# Autodesk Inventor assembly: Flash Hobby D3530 1100KV
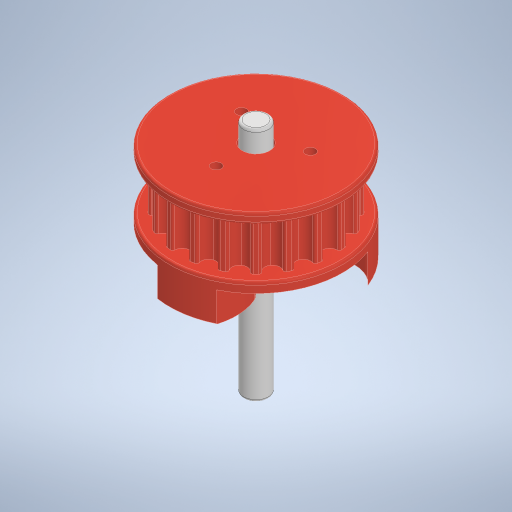
[picture p0: Inventor's stored thumbnail of the model, 512x512]
Saved by Autodesk Inventor 2023.2 (Build 272271000, 271)
## iProperties
Created: 2022-12-15
Part Number: Flash Hobby D3530 1100KV
Document SubType Name: Assembly
Designer: Nathan Cai
Author: Nathan Cai
## Documents named in this file (4)
- C:\Users\Nathan Cai\Documents\Inventor\Asorted Parts\Flash Hobby D3530 1100KV\Flash Hobby D3530 1100KV.iam
- C:\Users\Nathan Cai\Documents\Inventor\Asorted Parts\Flash Hobby D3530 1100KV\Body - Basic.ipt
- C:\Users\Nathan Cai\Documents\Inventor\Asorted Parts\Flash Hobby D3530 1100KV\Shaft.ipt
- C:\Users\Nathan Cai\Documents\Inventor\Asorted Parts\Flash Hobby D3530 1100KV\Simple_Vert4_weapon_pulley_orangeflash_v1\Simple_Vert4_weapon_pulley_orangeflash_v1.ipt
## Components (3 placed, 3 different names)
1. Body - Basic:1 — Mate:1, Flush:1, Mate:2, Mate:4
2. Shaft:1 — Mate:1, Flush:1, Mate:3
3. Simple_Vert4_weapon_pulley_orangeflash_v1:1 — Mate:2, Mate:3, Mate:4
## Relationships (5: Mate 4, Flush 1)
- Mate:1: Body - Basic:1 ↔ Shaft:1
- Flush:1 (-1.5 mm): Body - Basic:1 ↔ Shaft:1
- Mate:2: Body - Basic:1 ↔ Simple_Vert4_weapon_pulley_orangeflash_v1:1
- Mate:3: Shaft:1 ↔ Simple_Vert4_weapon_pulley_orangeflash_v1:1
- Mate:4: Body - Basic:1 ↔ Simple_Vert4_weapon_pulley_orangeflash_v1:1
